# Autodesk Inventor assembly: Hand
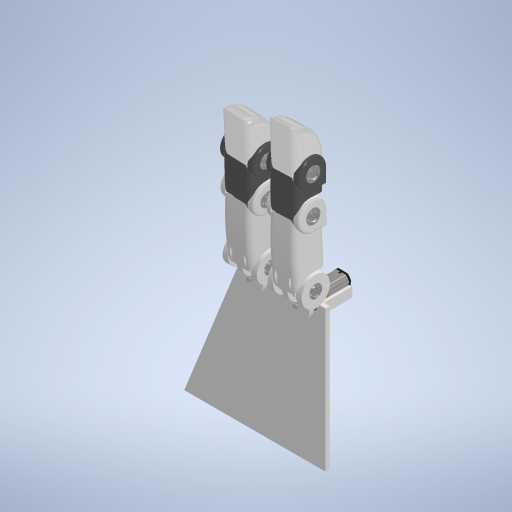
[picture p0: Inventor's stored thumbnail of the model, 512x512]
Saved by Autodesk Inventor 2024 (Build 280153000, 153)
## iProperties
Created: 2024-03-22
Part Number: Hand
Document SubType Name: Assembly
Designer: Wojtek
Author: Wojtek
## Documents named in this file (6)
- D:\STUDIA\inventor Projects\Bionic_Hand\Hand.iam
- D:\STUDIA\inventor Projects\Bionic_Hand\Fingers\KnuclePart.ipt
- D:\STUDIA\inventor Projects\Bionic_Hand\Fingers\BasePart.ipt
- D:\STUDIA\inventor Projects\motor_dc\Motor.iam
- C:\Users\Wojtek\OneDrive\Dokumenty\Inventor\Content Center Files\R2024\en-US\Bearing GB_T 292-2007\Rolling bearing B723 AC GB_T 292-2007.ipt
- D:\STUDIA\inventor Projects\Bionic_Hand\Fingers\Finger1.iam
## Components (11 placed, 5 different names)
1. KnuclePart:3 — Rotational:2, Rigid:3, Rotational:3
2. KnuclePart:4 — Rotational:1, Rigid:1, Rigid:2
3. BasePart:1 — Mate:1, Mate:2, Mate:3, Mate:4, Mate:5, Mate:6
4. GearMotor:1 [sub-assembly] — Mate:1, Mate:2, Rotational:1, Mate:3
5. GearMotor:2 [sub-assembly] — Mate:4, Mate:5, Mate:6, Rotational:2
6. Bearing GB/T 292-2007 Type IN - withdrawn B723 AC:1 — Rigid:1
7. Bearing GB/T 292-2007 Type IN - withdrawn B723 AC:2 — Rotational:3, Rotational:4
8. Bearing GB/T 292-2007 Type IN - withdrawn B723 AC:3 — Rigid:2, Rigid:4
9. Bearing GB/T 292-2007 Type IN - withdrawn B723 AC:4 — Rigid:3
10. Finger1:1 [sub-assembly] — Rigid:4
11. Finger1:2 [sub-assembly] — Rotational:4
## Relationships (14: Mate 6, RevoluteJoint 4, WeldJoint 4)
- Mate:1: BasePart:1 ↔ GearMotor:1
- Mate:2: BasePart:1 ↔ GearMotor:1
- Rotational:1 [RevoluteJoint] (-2 mm): KnuclePart:4 ↔ GearMotor:1
- Mate:3: BasePart:1 ↔ GearMotor:1
- Mate:4: BasePart:1 ↔ GearMotor:2
- Mate:5: BasePart:1 ↔ GearMotor:2
- Mate:6: BasePart:1 ↔ GearMotor:2
- Rotational:2 [RevoluteJoint] (-2 mm): KnuclePart:3 ↔ GearMotor:2
- Rigid:1 [WeldJoint] (-3.9 mm): KnuclePart:4 ↔ Bearing GB/T 292-2007 Type IN - withdrawn B723 AC:1
- Rigid:2 [WeldJoint] (-3.85 mm): KnuclePart:4 ↔ Bearing GB/T 292-2007 Type IN - withdrawn B723 AC:3
- Rigid:3 [WeldJoint] (-2 mm): KnuclePart:3 ↔ Bearing GB/T 292-2007 Type IN - withdrawn B723 AC:4
- Rotational:3 [RevoluteJoint] (-3.85 mm): KnuclePart:3 ↔ Bearing GB/T 292-2007 Type IN - withdrawn B723 AC:2
- Rotational:4 [RevoluteJoint] (-0.45 mm): Bearing GB/T 292-2007 Type IN - withdrawn B723 AC:2 ↔ Finger1:2
- Rigid:4 [WeldJoint] (0.6 mm): Bearing GB/T 292-2007 Type IN - withdrawn B723 AC:3 ↔ Finger1:1
